# Autodesk Inventor assembly: L3 Gearbox Assembly
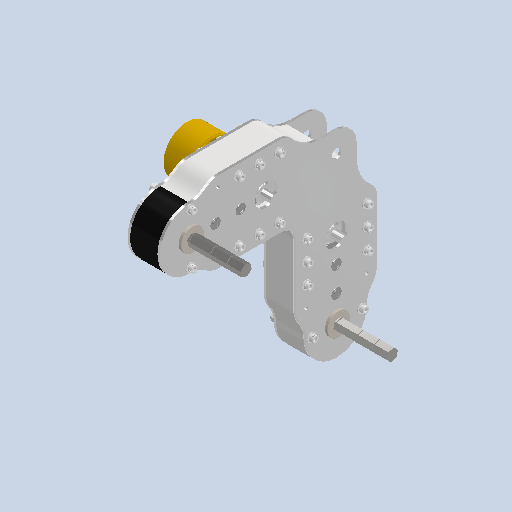
[picture p0: Inventor's stored thumbnail of the model, 512x512]
Saved by Autodesk Inventor 2025.1 (Build 291241020, 241B)
## iProperties
Created: 2023-02-14
Part Number: L3 Gearbox Assembly
Document SubType Name: Assembly
Designer: Dave
Mass: 1965.41 g
Surface Area: 3646.76 cm^2
Volume: 537.619 cm^3
Density: 3.65577 g/cm^3
Author: Dave
## Documents named in this file (16)
- C:\Users\t205b\OneDrive\Documents\Github\BehrendURCMechanical\CAD\Chassis V3\CH3-L3DoubleGearbox.iam
- C:\Users\t205b\OneDrive\Documents\Github\BehrendURCMechanical\CAD\Chassis V3\[Retired] GearBox\Final Gears and Assemblies\CH-1-01-20T_Drive Gear.ipt
- C:\Users\t205b\OneDrive\Documents\Github\BehrendURCMechanical\CAD\Chassis V3\[Retired] GearBox\Final Gears and Assemblies\CH-1-01-60T_Output.ipt
- C:\Users\t205b\OneDrive\Documents\Github\BehrendURCMechanical\CAD\Chassis V3\[Retired] GearBox\Final Gears and Assemblies\CH-1-01-20T_Idler.ipt
- C:\Users\t205b\OneDrive\Documents\Github\BehrendURCMechanical\CAD\Chassis V3\[Retired] GearBox\Final Gears and Assemblies\CH-1-01-60T_Idler.ipt
- C:\Users\t205b\OneDrive\Documents\Github\BehrendURCMechanical\CAD\Chassis V3\GearBox\Drive Motor Shaft Coupler.ipt
- C:\Users\t205b\OneDrive\Documents\Github\BehrendURCMechanical\CAD\Chassis V3\GearBox\Ch-1-01-0.5x4.5HexShaft.ipt
- C:\Users\t205b\OneDrive\Documents\Github\BehrendURCMechanical\CAD\Chassis V3\GearBox\CH-1-01-0.375x1.7TurnedHexShaft.ipt
- C:\Users\t205b\OneDrive\Documents\Github\BehrendURCMechanical\CAD\Chassis V3\GearBox\CH-1-01-0.5HexBearing.ipt
- C:\Users\t205b\OneDrive\Documents\Github\BehrendURCMechanical\CAD\Chassis V3\GearBox\CH-1-01-0.25IDSmoothBoreBearing.ipt
- C:\Users\t205b\OneDrive\Documents\Github\BehrendURCMechanical\CAD\Chassis V3\Hardware\91251A252_Black-Oxide Alloy Steel Socket Head Screw.ipt
- C:\Users\t205b\OneDrive\Documents\Github\BehrendURCMechanical\CAD\Chassis V3\Hardware\91831A011_18-8 Stainless Steel Nylon-Insert Locknut.ipt
- C:\Users\t205b\OneDrive\Documents\Github\BehrendURCMechanical\CAD\Chassis V3\Hardware\90107A011_316 Stainless Steel Washer.ipt
- C:\Users\t205b\OneDrive\Documents\Github\BehrendURCMechanical\CAD\Chassis V3\L3Plate.ipt
- C:\Users\t205b\OneDrive\Documents\Github\BehrendURCMechanical\CAD\Chassis V3\CH-L3GearboxCover.ipt
- C:\Users\t205b\OneDrive\Documents\Github\BehrendURCMechanical\CAD\Chassis V3\DriveMotorAssem\DriveMotorAssem.iam
## Components (101 placed, 15 different names)
1. L3Plate:1 — Insert:13, Insert:14, Insert:15, Insert:16, Insert:17, Insert:18, Insert:19, Insert:20, Flush:9, Mate:33, Mate:34, Mate:38, Mate:39, Mate:52
2. L3Plate:2 — Insert:39, Insert:41, Mate:35, Mate:41, Mate:52, Mate:56, Mate:57
3. CH-L3GearboxCover:1 — Mate:38, Mate:39, Mate:40, Mate:41
4. CH-1-01-0.25IDSmoothBoreBearing:4 — Mate:10, Mate:21
5. 90107A011_316 Stainless Steel Washer:2 — Insert:13, Insert:27
6. 90107A011_316 Stainless Steel Washer:3 — Insert:14, Insert:28
7. 90107A011_316 Stainless Steel Washer:5 — Insert:15, Insert:30
8. 90107A011_316 Stainless Steel Washer:7 — Insert:16, Insert:31
9. 90107A011_316 Stainless Steel Washer:9 — Insert:17, Insert:32
10. 90107A011_316 Stainless Steel Washer:15 — Insert:20, Insert:35
11. 90107A011_316 Stainless Steel Washer:13 — Insert:19, Insert:34
12. 90107A011_316 Stainless Steel Washer:11 — Insert:18, Insert:33
13. CH-1-01-60T_Output:1 — Mate:17, Flush:6
14. CH-1-01-20T_Idler:2 — Mate:19, Mate:22, Flush:6
15. CH-1-01-60T_Idler:1 — Mate:18, Mate:19, Flush:5, Mate:36
16. CH-1-01-20T_Idler:1 — Mate:21, Flush:5
17. CH-1-01-60T_Idler:2 — Mate:10, Mate:34
18. CH-1-01-20T_Drive Gear:1 — Mate:45, Mate:46
19. CH-1-01-0.5HexBearing:2 — Mate:8, Mate:9
20. CH-1-01-0.25IDSmoothBoreBearing:1 — Insert:12, Mate:33
21. CH-1-01-0.375x1.7TurnedHexShaft:1 — Mate:32, Flush:9
22. CH-1-01-0.25IDSmoothBoreBearing:2 — Mate:32
23. Drive Motor Shaft Coupler:1 — Mate:45, Mate:46, Mate:54, Mate:58
24. CH-1-01-0.375x1.7TurnedHexShaft:2 — Insert:12
25. CH-1-01-0.25IDSmoothBoreBearing:3 — Mate:18, Mate:22, Mate:36
26. Ch-1-01-0.5x4.5HexShaft:1 — Mate:8, Mate:9, Flush:8
27. CH-1-01-0.5HexBearing:1 — Mate:17, Flush:8
28. 90107A011_316 Stainless Steel Washer:8 — Insert:39, Insert:45
29. 91831A011_18-8 Stainless Steel Nylon-Insert Locknut:1 — Insert:45
30. 91251A252_Black-Oxide Alloy Steel Socket Head Screw:3 — Insert:31
31. 90107A011_316 Stainless Steel Washer:10 — Insert:40, Insert:41
32. 91831A011_18-8 Stainless Steel Nylon-Insert Locknut:7 — Insert:40
33. 91251A252_Black-Oxide Alloy Steel Socket Head Screw:4 — Insert:32
34. 90107A011_316 Stainless Steel Washer:16 — Insert:44, Mate:67
35. 91831A011_18-8 Stainless Steel Nylon-Insert Locknut:8 — Insert:44, Mate:64
36. 91251A252_Black-Oxide Alloy Steel Socket Head Screw:8 — Insert:35, Mate:64
37. 90107A011_316 Stainless Steel Washer:14 — Insert:43, Mate:66
38. 91831A011_18-8 Stainless Steel Nylon-Insert Locknut:6 — Insert:43, Mate:65
39. 91251A252_Black-Oxide Alloy Steel Socket Head Screw:7 — Insert:34, Mate:65
40. 90107A011_316 Stainless Steel Washer:12 — Mate:35
41. 91831A011_18-8 Stainless Steel Nylon-Insert Locknut:5 — Mate:68, Mate:69
42. 91251A252_Black-Oxide Alloy Steel Socket Head Screw:6 — Insert:33, Mate:68
43. 91831A011_18-8 Stainless Steel Nylon-Insert Locknut:2 — Insert:38, Mate:51
44. 91251A252_Black-Oxide Alloy Steel Socket Head Screw:5 — Insert:30, Mate:51
45. 90107A011_316 Stainless Steel Washer:6 — Insert:38, Mate:63
46. 91251A252_Black-Oxide Alloy Steel Socket Head Screw:2 — Insert:28, Mate:40, Mate:61
47. 90107A011_316 Stainless Steel Washer:4 — Insert:37, Mate:62
48. 91831A011_18-8 Stainless Steel Nylon-Insert Locknut:3 — Insert:37, Mate:61
49. 90107A011_316 Stainless Steel Washer:1 — Insert:36, Mate:60
50. 91251A252_Black-Oxide Alloy Steel Socket Head Screw:1 — Insert:27, Mate:55, Mate:59
51. 91831A011_18-8 Stainless Steel Nylon-Insert Locknut:4 — Insert:36, Mate:59
52. DriveMotorAssem:1 [sub-assembly] — Mate:54, Mate:55, Mate:56, Mate:57, Mate:58, Mate:60, Mate:62, Mate:63, Mate:66, Mate:67, Mate:69
53. CH-1-01-0.25IDSmoothBoreBearing:5
54. 90107A011_316 Stainless Steel Washer:17
55. 90107A011_316 Stainless Steel Washer:18
56. 90107A011_316 Stainless Steel Washer:19
57. 90107A011_316 Stainless Steel Washer:20
58. 90107A011_316 Stainless Steel Washer:21
59. 90107A011_316 Stainless Steel Washer:22
60. 90107A011_316 Stainless Steel Washer:23
61. 90107A011_316 Stainless Steel Washer:24
62. CH-1-01-60T_Output:2
63. CH-1-01-20T_Idler:3
64. CH-1-01-60T_Idler:3
65. CH-1-01-20T_Idler:4
66. CH-1-01-60T_Idler:4
67. CH-1-01-20T_Drive Gear:2
68. CH-1-01-0.5HexBearing:3
69. CH-1-01-0.25IDSmoothBoreBearing:6
70. CH-1-01-0.375x1.7TurnedHexShaft:3
71. CH-1-01-0.25IDSmoothBoreBearing:7
72. Drive Motor Shaft Coupler:2
73. CH-1-01-0.375x1.7TurnedHexShaft:4
74. CH-1-01-0.25IDSmoothBoreBearing:8
75. Ch-1-01-0.5x4.5HexShaft:2
76. CH-1-01-0.5HexBearing:4
77. 90107A011_316 Stainless Steel Washer:25
78. 91831A011_18-8 Stainless Steel Nylon-Insert Locknut:9
79. 91251A252_Black-Oxide Alloy Steel Socket Head Screw:9
80. 90107A011_316 Stainless Steel Washer:26
81. 91831A011_18-8 Stainless Steel Nylon-Insert Locknut:10
82. 91251A252_Black-Oxide Alloy Steel Socket Head Screw:10
83. 90107A011_316 Stainless Steel Washer:27
84. 91831A011_18-8 Stainless Steel Nylon-Insert Locknut:11
85. 91251A252_Black-Oxide Alloy Steel Socket Head Screw:11
86. 90107A011_316 Stainless Steel Washer:28
87. 91831A011_18-8 Stainless Steel Nylon-Insert Locknut:12
88. 91251A252_Black-Oxide Alloy Steel Socket Head Screw:12
89. 90107A011_316 Stainless Steel Washer:29
90. 91831A011_18-8 Stainless Steel Nylon-Insert Locknut:13
91. 91251A252_Black-Oxide Alloy Steel Socket Head Screw:13
92. 91831A011_18-8 Stainless Steel Nylon-Insert Locknut:14
93. 91251A252_Black-Oxide Alloy Steel Socket Head Screw:14
94. 90107A011_316 Stainless Steel Washer:30
95. 91251A252_Black-Oxide Alloy Steel Socket Head Screw:15
96. 90107A011_316 Stainless Steel Washer:31
97. 91831A011_18-8 Stainless Steel Nylon-Insert Locknut:15
98. 90107A011_316 Stainless Steel Washer:32
99. 91251A252_Black-Oxide Alloy Steel Socket Head Screw:16
100. 91831A011_18-8 Stainless Steel Nylon-Insert Locknut:16
101. DriveMotorAssem:2 [sub-assembly]
## Component patterns: (2 elements, first: CH-1-01-0.25IDSmoothBoreBearing:4 + 90107A011_316 Stainless Steel Washer:2 + 90107A011_316 Stainless Steel Washer:3 + 90107A011_316 Stainless Steel Washer:5 + 90107A011_316 Stainless Steel Washer:7 + 90107A011_316 Stainless Steel Washer:9 + 90107A011_316 Stainless Steel Washer:15 + 90107A011_316 Stainless Steel Washer:13 + 90107A011_316 Stainless Steel Washer:11 + CH-1-01-60T_Output:1 + CH-1-01-20T_Idler:2 + CH-1-01-60T_Idler:1 + CH-1-01-20T_Idler:1 + CH-1-01-60T_Idler:2 + CH-1-01-20T_Drive Gear:1 + CH-1-01-0.5HexBearing:2 + CH-1-01-0.25IDSmoothBoreBearing:1 + CH-1-01-0.375x1.7TurnedHexShaft:1 + CH-1-01-0.25IDSmoothBoreBearing:2 + Drive Motor Shaft Coupler:1 + CH-1-01-0.375x1.7TurnedHexShaft:2 + CH-1-01-0.25IDSmoothBoreBearing:3 + Ch-1-01-0.5x4.5HexShaft:1 + CH-1-01-0.5HexBearing:1 + 90107A011_316 Stainless Steel Washer:8 + 91831A011_18-8 Stainless Steel Nylon-Insert Locknut:1 + 91251A252_Black-Oxide Alloy Steel Socket Head Screw:3 + 90107A011_316 Stainless Steel Washer:10 + 91831A011_18-8 Stainless Steel Nylon-Insert Locknut:7 + 91251A252_Black-Oxide Alloy Steel Socket Head Screw:4 + 90107A011_316 Stainless Steel Washer:16 + 91831A011_18-8 Stainless Steel Nylon-Insert Locknut:8 + 91251A252_Black-Oxide Alloy Steel Socket Head Screw:8 + 90107A011_316 Stainless Steel Washer:14 + 91831A011_18-8 Stainless Steel Nylon-Insert Locknut:6 + 91251A252_Black-Oxide Alloy Steel Socket Head Screw:7 + 90107A011_316 Stainless Steel Washer:12 + 91831A011_18-8 Stainless Steel Nylon-Insert Locknut:5 + 91251A252_Black-Oxide Alloy Steel Socket Head Screw:6 + 91831A011_18-8 Stainless Steel Nylon-Insert Locknut:2 + 91251A252_Black-Oxide Alloy Steel Socket Head Screw:5 + 90107A011_316 Stainless Steel Washer:6 + 91251A252_Black-Oxide Alloy Steel Socket Head Screw:2 + 90107A011_316 Stainless Steel Washer:4 + 91831A011_18-8 Stainless Steel Nylon-Insert Locknut:3 + 90107A011_316 Stainless Steel Washer:1 + 91251A252_Black-Oxide Alloy Steel Socket Head Screw:1 + 91831A011_18-8 Stainless Steel Nylon-Insert Locknut:4 + DriveMotorAssem:1)
## Relationships (75: Mate 37, Insert 32, Flush 5, Angle 1)
- [Angle] (0 deg): L3Plate:1
- [Flush]: L3Plate:1 ↔ L3Plate:2
- [Insert]: L3Plate:1 ↔ CH-1-01-0.25IDSmoothBoreBearing:1
- [Insert]: L3Plate:1 ↔ CH-1-01-0.25IDSmoothBoreBearing:2
- [Insert]: L3Plate:2 ↔ CH-1-01-0.25IDSmoothBoreBearing:3
- [Insert]: L3Plate:2 ↔ CH-1-01-0.25IDSmoothBoreBearing:4
- [Insert]: L3Plate:1 ↔ CH-1-01-0.5HexBearing:2
- [Insert]: L3Plate:2 ↔ CH-1-01-0.5HexBearing:1
- Mate:8: CH-1-01-0.5HexBearing:2 ↔ Ch-1-01-0.5x4.5HexShaft:1
- Mate:9: CH-1-01-0.5HexBearing:2 ↔ Ch-1-01-0.5x4.5HexShaft:1
- Insert:12: CH-1-01-0.25IDSmoothBoreBearing:1 ↔ CH-1-01-0.375x1.7TurnedHexShaft:2
- Mate:10: CH-1-01-0.25IDSmoothBoreBearing:4 ↔ CH-1-01-60T_Idler:2
- Mate:17: CH-1-01-60T_Output:1 ↔ CH-1-01-0.5HexBearing:1
- Mate:18: CH-1-01-60T_Idler:1 ↔ CH-1-01-0.25IDSmoothBoreBearing:3
- Mate:19: CH-1-01-20T_Idler:2 ↔ CH-1-01-60T_Idler:1
- Mate:21: CH-1-01-0.25IDSmoothBoreBearing:4 ↔ CH-1-01-20T_Idler:1
- Flush:5: CH-1-01-60T_Idler:1 ↔ CH-1-01-20T_Idler:1
- Mate:22: CH-1-01-20T_Idler:2 ↔ CH-1-01-0.25IDSmoothBoreBearing:3
- Flush:6: CH-1-01-60T_Output:1 ↔ CH-1-01-20T_Idler:2
- Flush:8: Ch-1-01-0.5x4.5HexShaft:1 ↔ CH-1-01-0.5HexBearing:1
- Insert:13: L3Plate:1 ↔ 90107A011_316 Stainless Steel Washer:2
- Insert:14: L3Plate:1 ↔ 90107A011_316 Stainless Steel Washer:3
- Insert:15: L3Plate:1 ↔ 90107A011_316 Stainless Steel Washer:5
- Insert:16: L3Plate:1 ↔ 90107A011_316 Stainless Steel Washer:7
- Insert:17: L3Plate:1 ↔ 90107A011_316 Stainless Steel Washer:9
- Insert:18: L3Plate:1 ↔ 90107A011_316 Stainless Steel Washer:11
- Insert:19: L3Plate:1 ↔ 90107A011_316 Stainless Steel Washer:13
- Insert:20: L3Plate:1 ↔ 90107A011_316 Stainless Steel Washer:15
- Insert:27: 90107A011_316 Stainless Steel Washer:2 ↔ 91251A252_Black-Oxide Alloy Steel Socket Head Screw:1
- Insert:28: 90107A011_316 Stainless Steel Washer:3 ↔ 91251A252_Black-Oxide Alloy Steel Socket Head Screw:2
- Insert:30: 90107A011_316 Stainless Steel Washer:5 ↔ 91251A252_Black-Oxide Alloy Steel Socket Head Screw:5
- Insert:31: 90107A011_316 Stainless Steel Washer:7 ↔ 91251A252_Black-Oxide Alloy Steel Socket Head Screw:3
- Insert:32: 90107A011_316 Stainless Steel Washer:9 ↔ 91251A252_Black-Oxide Alloy Steel Socket Head Screw:4
- Insert:33: 90107A011_316 Stainless Steel Washer:11 ↔ 91251A252_Black-Oxide Alloy Steel Socket Head Screw:6
- Insert:34: 90107A011_316 Stainless Steel Washer:13 ↔ 91251A252_Black-Oxide Alloy Steel Socket Head Screw:7
- Insert:35: 90107A011_316 Stainless Steel Washer:15 ↔ 91251A252_Black-Oxide Alloy Steel Socket Head Screw:8
- Insert:36: 90107A011_316 Stainless Steel Washer:1 ↔ 91831A011_18-8 Stainless Steel Nylon-Insert Locknut:4
- Insert:37: 90107A011_316 Stainless Steel Washer:4 ↔ 91831A011_18-8 Stainless Steel Nylon-Insert Locknut:3
- Insert:38: 91831A011_18-8 Stainless Steel Nylon-Insert Locknut:2 ↔ 90107A011_316 Stainless Steel Washer:6
- Insert:39: L3Plate:2 ↔ 90107A011_316 Stainless Steel Washer:8
- Insert:40: 90107A011_316 Stainless Steel Washer:10 ↔ 91831A011_18-8 Stainless Steel Nylon-Insert Locknut:7
- Insert:41: L3Plate:2 ↔ 90107A011_316 Stainless Steel Washer:10
- Insert:43: 90107A011_316 Stainless Steel Washer:14 ↔ 91831A011_18-8 Stainless Steel Nylon-Insert Locknut:6
- Insert:44: 90107A011_316 Stainless Steel Washer:16 ↔ 91831A011_18-8 Stainless Steel Nylon-Insert Locknut:8
- Insert:45: 90107A011_316 Stainless Steel Washer:8 ↔ 91831A011_18-8 Stainless Steel Nylon-Insert Locknut:1
- Mate:32: CH-1-01-0.375x1.7TurnedHexShaft:1 ↔ CH-1-01-0.25IDSmoothBoreBearing:2
- Flush:9: L3Plate:1 ↔ CH-1-01-0.375x1.7TurnedHexShaft:1
- Mate:33: L3Plate:1 ↔ CH-1-01-0.25IDSmoothBoreBearing:1
- Mate:34: L3Plate:1 ↔ CH-1-01-60T_Idler:2
- Mate:35: L3Plate:2 ↔ 90107A011_316 Stainless Steel Washer:12
- Mate:36: CH-1-01-60T_Idler:1 ↔ CH-1-01-0.25IDSmoothBoreBearing:3
- Mate:38: L3Plate:1 ↔ CH-L3GearboxCover:1
- Mate:39: L3Plate:1 ↔ CH-L3GearboxCover:1
- Mate:40: CH-L3GearboxCover:1 ↔ 91251A252_Black-Oxide Alloy Steel Socket Head Screw:2
- Mate:41: L3Plate:2 ↔ CH-L3GearboxCover:1
- Mate:45: CH-1-01-20T_Drive Gear:1 ↔ Drive Motor Shaft Coupler:1
- Mate:46: CH-1-01-20T_Drive Gear:1 ↔ Drive Motor Shaft Coupler:1
- Mate:51: 91831A011_18-8 Stainless Steel Nylon-Insert Locknut:2 ↔ 91251A252_Black-Oxide Alloy Steel Socket Head Screw:5
- Mate:52: L3Plate:1 ↔ L3Plate:2
- Mate:54: Drive Motor Shaft Coupler:1 ↔ DriveMotorAssem:1
- Mate:55: 91251A252_Black-Oxide Alloy Steel Socket Head Screw:1 ↔ DriveMotorAssem:1
- Mate:56: L3Plate:2 ↔ DriveMotorAssem:1
- Mate:57: L3Plate:2 ↔ DriveMotorAssem:1
- Mate:58: Drive Motor Shaft Coupler:1 ↔ DriveMotorAssem:1
- Mate:59: 91251A252_Black-Oxide Alloy Steel Socket Head Screw:1 ↔ 91831A011_18-8 Stainless Steel Nylon-Insert Locknut:4
- Mate:60: 90107A011_316 Stainless Steel Washer:1 ↔ DriveMotorAssem:1
- Mate:61: 91251A252_Black-Oxide Alloy Steel Socket Head Screw:2 ↔ 91831A011_18-8 Stainless Steel Nylon-Insert Locknut:3
- Mate:62: 90107A011_316 Stainless Steel Washer:4 ↔ DriveMotorAssem:1
- Mate:63: 90107A011_316 Stainless Steel Washer:6 ↔ DriveMotorAssem:1
- Mate:64: 91831A011_18-8 Stainless Steel Nylon-Insert Locknut:8 ↔ 91251A252_Black-Oxide Alloy Steel Socket Head Screw:8
- Mate:65: 91831A011_18-8 Stainless Steel Nylon-Insert Locknut:6 ↔ 91251A252_Black-Oxide Alloy Steel Socket Head Screw:7
- Mate:66: 90107A011_316 Stainless Steel Washer:14 ↔ DriveMotorAssem:1
- Mate:67: 90107A011_316 Stainless Steel Washer:16 ↔ DriveMotorAssem:1
- Mate:68: 91831A011_18-8 Stainless Steel Nylon-Insert Locknut:5 ↔ 91251A252_Black-Oxide Alloy Steel Socket Head Screw:6
- Mate:69: 91831A011_18-8 Stainless Steel Nylon-Insert Locknut:5 ↔ DriveMotorAssem:1
